# Autodesk Inventor assembly: SinglePulley
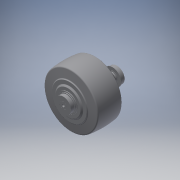
[picture p0: Inventor's stored thumbnail of the model, 180x180]
Saved by Autodesk Inventor 2016 (Build 200138000, 138)
## iProperties
Created: 2017-01-15
Part Number: SinglePulley
Document SubType Name: Assembly
Designer: Kyle
Author: Kyle
## Documents named in this file (6)
- F:\FRC\2017\DriveTrainRev3\Individual Parts\SinglePulley.iam
- F:\FRC\2017\DriveTrainRev3\Individual Parts\.5Bearing.ipt
- F:\FRC\2017\DriveTrainRev3\Individual Parts\4x2Colson.ipt
- F:\FRC\2017\DriveTrainRev3\Individual Parts\24t9MMPulley6mm.ipt
- F:\FRC\2017\DriveTrainRev3\Individual Parts\.441Spacer.ipt
- F:\FRC\2017\DriveTrainRev3\Individual Parts\.5HexShaft3.875in.ipt
## Components (7 placed, 5 different names)
1. .5Bearing:1 — Mate:3, Mate:20, Flush:2
2. 4x2Colson:1 — Mate:3, Mate:11
3. 24t9MMPulley6mm:1 — Mate:11, Mate:16, Mate:17
4. .5Bearing:2 — Mate:19
5. 24t9MMPulley6mm:2 — Mate:16, Mate:17
6. .441Spacer:1 — Mate:19
7. .5HexShaft3.875in:1 — Mate:20, Flush:2
## Relationships (7: Mate 6, Flush 1)
- Mate:3: .5Bearing:1 ↔ 4x2Colson:1
- Mate:11: 4x2Colson:1 ↔ 24t9MMPulley6mm:1
- Mate:16: 24t9MMPulley6mm:1 ↔ 24t9MMPulley6mm:2
- Mate:17: 24t9MMPulley6mm:1 ↔ 24t9MMPulley6mm:2
- Mate:19: .5Bearing:2 ↔ .441Spacer:1
- Mate:20: .5Bearing:1 ↔ .5HexShaft3.875in:1
- Flush:2: .5Bearing:1 ↔ .5HexShaft3.875in:1
